# Autodesk Inventor assembly: SCARA M1
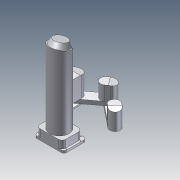
[picture p0: Inventor's stored thumbnail of the model, 180x180]
Saved by Autodesk Inventor 2011 (Build 150239000, 239)
## iProperties
Category: TPA
Manager: BỘ
Company: TPA
Created: 2018-01-17
Part Number: SCARA M1
Project: 419
Document SubType Name: Assembly
Designer: tuan.bt
Mass: 12318.3 g
Surface Area: 7319.43 cm^2
Volume: 16894.8 cm^3
Density: 0.729116 g/cm^3
Author: tuan.bt
## Documents named in this file (5)
- C:\Users\Administrator.HauTk2TPA-PC\Desktop\DOBOT\SCARA M1.iam
- C:\Users\Administrator.HauTk2TPA-PC\Desktop\DOBOT\THAN M1.ipt
- C:\Users\Administrator.HauTk2TPA-PC\Desktop\DOBOT\CANH TAY 1.ipt
- C:\Users\Administrator.HauTk2TPA-PC\Desktop\DOBOT\CANH TAY 2.ipt
- C:\Users\Administrator.HauTk2TPA-PC\Desktop\DOBOT\CANH TAY 3.ipt
## Components (4 placed, 4 different names)
1. THAN M1:1 — Mate:3
2. CANH TAY 1:1 — Mate:3, Mate:4, Insert:1
3. CANH TAY 2:1 — Insert:1, Insert:2
4. CANH TAY 3:1 — Insert:2
## Relationships (4: Mate 2, Insert 2)
- Mate:3 (123 mm): THAN M1:1 ↔ CANH TAY 1:1
- Mate:4: CANH TAY 1:1
- Insert:1: CANH TAY 1:1 ↔ CANH TAY 2:1
- Insert:2: CANH TAY 2:1 ↔ CANH TAY 3:1
